# Autodesk Inventor assembly: CATIA用
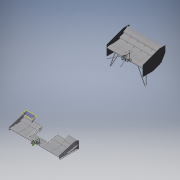
[picture p0: Inventor's stored thumbnail of the model, 180x180]
Saved by Autodesk Inventor 2018 (Build 220112000, 112)
## iProperties
Created: 2018-03-12
Part Number: CATIA用
Material: 一般
Document SubType Name: Assembly
Designer: ku_sk
Author: ku_sk
## Documents named in this file (3)
- D:\Users\ku_sk\Documents\Inventor\Aero\KS-15\CATIA用.iam
- D:\Users\ku_sk\Documents\Inventor\Aero\KS-15\Fr.wing\Fr.wing_assy.iam
- D:\Users\ku_sk\Documents\Inventor\Aero\KS-15\Rr.wing\Rr.wing_assy.iam
## Components (2 placed, 2 different names)
1. Fr.wing_assy:1 [sub-assembly] — フラッシュ:1
2. Rr.wing_assy:1 [sub-assembly] — フラッシュ:6, フラッシュ:7, フラッシュ:8
## Relationships (4: Flush 4)
- フラッシュ:1 [Flush]: Fr.wing_assy:1
- フラッシュ:6 [Flush]: Rr.wing_assy:1
- フラッシュ:7 [Flush] (460 mm): Rr.wing_assy:1
- フラッシュ:8 [Flush] (-1080 mm): Rr.wing_assy:1
